# Autodesk Inventor assembly: Respirator
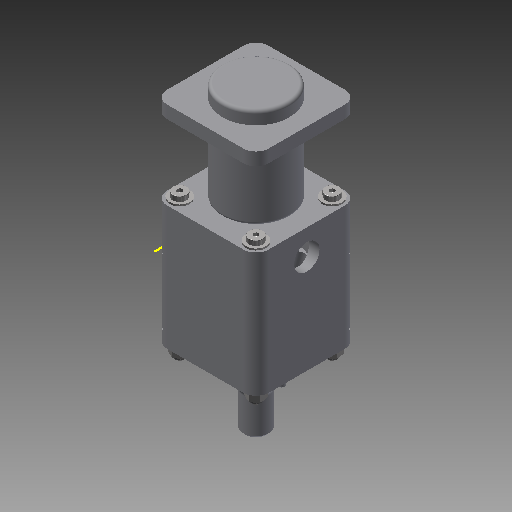
[picture p0: Inventor's stored thumbnail of the model, 512x512]
Saved by Autodesk Inventor 2018 (Build 220112000, 112)
## iProperties
Created: 2020-03-23
Part Number: Respirator
Document SubType Name: Assembly
Designer: emile
Author: emile
## Documents named in this file (13)
- C:\Users\emile\OneDrive\Documents\Inventor\Respirator\Respirator.iam
- C:\Users\emile\OneDrive\Documents\Inventor\Respirator\frame.ipt
- C:\Users\emile\OneDrive\Documents\Inventor\Respirator\McMaster60355K430_BALL BEARING.ipt
- C:\Users\emile\OneDrive\Documents\Inventor\Content Center Files\R2018\en-US\ANSI B18.22.1\ANSI B18.22.1 - 1_4 - narrow - Type B.ipt
- C:\Users\emile\OneDrive\Documents\Inventor\Respirator\Fan.ipt
- C:\Users\emile\OneDrive\Documents\Inventor\Respirator\FrameToPipe.ipt
- C:\Users\emile\OneDrive\Documents\Inventor\Respirator\Respirator\Design Accelerator\Bolted Connection2.iam
- C:\Users\emile\OneDrive\Documents\Inventor\Content Center Files\R2018\en-US\ANSI B18.2.2(09)\ANSI B18.2.2 - 1_4 - 20(2).ipt
- C:\Users\emile\OneDrive\Documents\Inventor\Respirator\DC Brush Motor 24V 150W High Speed Motor with Belt Pulley for DIY Generator Electric Vehicle Motor.ipt
- C:\Users\emile\OneDrive\Documents\Inventor\Respirator\Crabot 1-4 to 11-32.iam
- C:\Users\emile\OneDrive\Documents\Inventor\Respirator\Air Zone.ipt
- C:\Users\emile\OneDrive\Documents\Inventor\Respirator\Respirator\Design Accelerator\Bolted Connection3.iam
- C:\Users\emile\OneDrive\Documents\Inventor\Respirator\MotorBlock.ipt
## Components (18 placed, 11 different names)
1. frame:1 — Mate:1, Mate:2, Flush:2, Flush:3, Flush:4, Mate:15, Mate:18, Flush:5, Mate:45, Mate:46, Flush:6
2. McMaster60355K430_BALL BEARING:1 — Mate:1, Mate:2, Insert:1, Mate:3, Mate:4
3. Plain Washer (Inch) 1/4 - narrow - Type B:1 — Insert:1, Mate:5
4. Plain Washer (Inch) 1/4 - narrow - Type B:2 — Mate:3, Mate:4, Mate:34, Mate:40
5. Fan:1 — Mate:5, Mate:7, Mate:8, Mate:15, Mate:19, Mate:51, Mate:52
6. Plain Washer (Inch) 1/4 - narrow - Type B:3 — Mate:7, Mate:8
7. FrameToPipe:1 — Mate:16, Mate:17, Mate:18, Mate:19, Flush:5
8. McMaster60355K430_BALL BEARING:2 — Mate:13, Mate:14, Mate:16, Mate:17
9. Plain Washer (Inch) 1/4 - narrow - Type B:4 — Mate:13, Mate:14, Mate:39
10. Bolted Connection:1 [sub-assembly] — Mate:39, Mate:40, Mate:41, Mate:42, Mate:43, Mate:53
11. Hex Nut - Inch 1/4 - 20:1 — Mate:36, Mate:42
12. DC Brush Motor 24V 150W High Speed Motor with Belt Pulley for DIY Generator Electric Vehicle Motor:1 — Mate:44, Mate:47, Mate:48, Mate:56, Flush:8
13. Crabot 1-4 to 11-32:1 [sub-assembly] — Mate:41, Mate:43, Mate:44
14. Plain Washer (Inch) 1/4 - narrow - Type B:5 — Mate:34, Mate:36
15. Air Zone:1 — Mate:45, Mate:46, Flush:6, Mate:47, Mate:48, Mate:54, Mate:55, Flush:7
16. Bolted Connection:2 [sub-assembly] — Mate:54, Mate:55
17. Hex Nut - Inch 1/4 - 20:2 — Mate:51, Mate:52, Mate:53
18. MotorBlock:1 — Mate:56, Flush:7, Flush:8
## Relationships (40: Mate 32, Flush 7, Insert 1)
- Mate:1: frame:1 ↔ McMaster60355K430_BALL BEARING:1
- Mate:2: frame:1 ↔ McMaster60355K430_BALL BEARING:1
- Flush:2: frame:1
- Flush:3: frame:1
- Insert:1: McMaster60355K430_BALL BEARING:1 ↔ Plain Washer (Inch) 1/4 - narrow - Type B:1
- Mate:3: McMaster60355K430_BALL BEARING:1 ↔ Plain Washer (Inch) 1/4 - narrow - Type B:2
- Mate:4: McMaster60355K430_BALL BEARING:1 ↔ Plain Washer (Inch) 1/4 - narrow - Type B:2
- Mate:5: Plain Washer (Inch) 1/4 - narrow - Type B:1 ↔ Fan:1
- Mate:7: Fan:1 ↔ Plain Washer (Inch) 1/4 - narrow - Type B:3
- Mate:8: Fan:1 ↔ Plain Washer (Inch) 1/4 - narrow - Type B:3
- Mate:13: McMaster60355K430_BALL BEARING:2 ↔ Plain Washer (Inch) 1/4 - narrow - Type B:4
- Mate:14: McMaster60355K430_BALL BEARING:2 ↔ Plain Washer (Inch) 1/4 - narrow - Type B:4
- Flush:4: frame:1
- Mate:15: frame:1 ↔ Fan:1
- Mate:16: FrameToPipe:1 ↔ McMaster60355K430_BALL BEARING:2
- Mate:17: FrameToPipe:1 ↔ McMaster60355K430_BALL BEARING:2
- Mate:18: frame:1 ↔ FrameToPipe:1
- Mate:19: Fan:1 ↔ FrameToPipe:1
- Flush:5: frame:1 ↔ FrameToPipe:1
- Mate:34: Plain Washer (Inch) 1/4 - narrow - Type B:2 ↔ Plain Washer (Inch) 1/4 - narrow - Type B:5
- Mate:36: Hex Nut - Inch 1/4 - 20:1 ↔ Plain Washer (Inch) 1/4 - narrow - Type B:5
- Mate:39: Plain Washer (Inch) 1/4 - narrow - Type B:4 ↔ Bolted Connection:1
- Mate:40: Plain Washer (Inch) 1/4 - narrow - Type B:2 ↔ Bolted Connection:1
- Mate:41: Bolted Connection:1 ↔ Crabot 1-4 to 11-32:1
- Mate:42: Bolted Connection:1 ↔ Hex Nut - Inch 1/4 - 20:1
- Mate:43: Bolted Connection:1 ↔ Crabot 1-4 to 11-32:1
- Mate:44: DC Brush Motor 24V 150W High Speed Motor with Belt Pulley for DIY Generator Electric Vehicle Motor:1 ↔ Crabot 1-4 to 11-32:1
- Mate:45: frame:1 ↔ Air Zone:1
- Mate:46: frame:1 ↔ Air Zone:1
- Flush:6: frame:1 ↔ Air Zone:1
- Mate:47: DC Brush Motor 24V 150W High Speed Motor with Belt Pulley for DIY Generator Electric Vehicle Motor:1 ↔ Air Zone:1
- Mate:48: DC Brush Motor 24V 150W High Speed Motor with Belt Pulley for DIY Generator Electric Vehicle Motor:1 ↔ Air Zone:1
- Mate:51: Fan:1 ↔ Hex Nut - Inch 1/4 - 20:2
- Mate:52: Fan:1 ↔ Hex Nut - Inch 1/4 - 20:2
- Mate:53: Bolted Connection:1 ↔ Hex Nut - Inch 1/4 - 20:2
- Mate:54: Air Zone:1 ↔ Bolted Connection:2
- Mate:55: Air Zone:1 ↔ Bolted Connection:2
- Mate:56: DC Brush Motor 24V 150W High Speed Motor with Belt Pulley for DIY Generator Electric Vehicle Motor:1 ↔ MotorBlock:1
- Flush:7: Air Zone:1 ↔ MotorBlock:1
- Flush:8 (12.7 mm): DC Brush Motor 24V 150W High Speed Motor with Belt Pulley for DIY Generator Electric Vehicle Motor:1 ↔ MotorBlock:1
